# Autodesk Inventor assembly: Assembly2
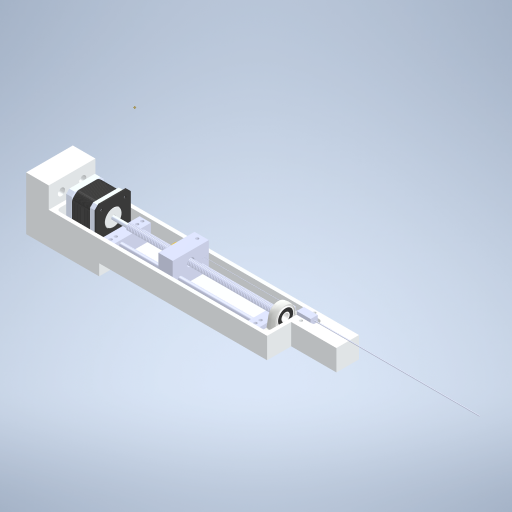
[picture p0: Inventor's stored thumbnail of the model, 512x512]
Saved by Autodesk Inventor 2023 (Build 270158000, 158)
## iProperties
Created: 2023-02-17
Part Number: Assembly2
Document SubType Name: Assembly
Designer: klebe
Author: klebe
## Documents named in this file (2)
- C:\Users\klebe\OneDrive\Documents\GitHub\Sala-braquiterapia\Sala de Braquiterapia\Inventor\Mateus]\Ferramenta Braquiterapia Solid\Assembly2.iam
- C:\Users\klebe\OneDrive\Documents\GitHub\Sala-braquiterapia\Sala de Braquiterapia\Inventor\Mateus]\Ferramenta Braquiterapia Solid\MontagemFerramentaTCC2.iam
## Components (1 placed, 1 different names)
1. MontagemFerramentaTCC2:1 [sub-assembly] — Flush:1, Mate:1, Mate:2
## Relationships (3: Mate 2, Flush 1)
- Flush:1: MontagemFerramentaTCC2:1
- Mate:1: MontagemFerramentaTCC2:1
- Mate:2: MontagemFerramentaTCC2:1
